# Autodesk Inventor assembly: MeasurementChamber RollBase V1
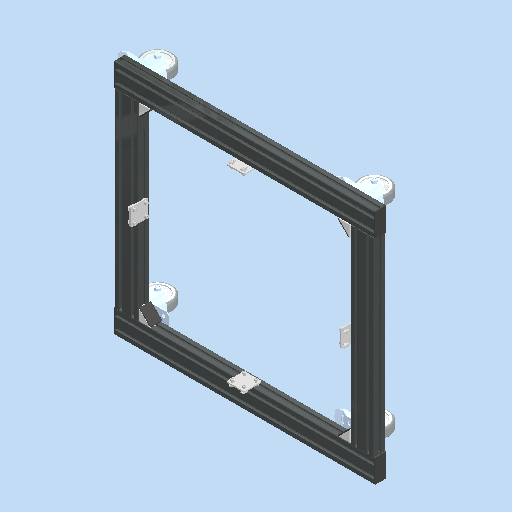
[picture p0: Inventor's stored thumbnail of the model, 512x512]
Saved by Autodesk Inventor 2023.2 (Build 272271000, 271)
## iProperties
Created: 2024-02-20
Part Number: MeasurementChamber RollBase V1
Document SubType Name: Assembly
Designer: Nils Bade
Author: Nils Bade
## Documents named in this file (10)
- C:\Users\nilsb\Documents\Inventor\Projektarbeit-Bade\RatRig_Bade\MeasurementChamber RollBase V1.iam
- C:\Users\nilsb\Documents\Inventor\Projektarbeit-Bade\ITEM\4040 Profile\ITEM T-SLOT 8040 875mm_65530.ipt
- C:\Users\nilsb\Documents\Inventor\Projektarbeit-Bade\ITEM\ITEM_41115_Winkelsatz_90er.iam
- C:\Users\nilsb\Documents\Inventor\Projektarbeit-Bade\ITEM\ITEM Bausätze\ITEM_66718_Lenkrolle-d100-doppelfest.iam
- ITEM_66718_Lenkrolle-d100-doppelfest.iam
- C:\Users\nilsb\Documents\Inventor\Projektarbeit-Bade\ITEM\ITEM Bausätze\ITEM_67018_Befestigungssatz.iam
- ITEM_Befestigungssatz_67018.iam
- C:\Users\nilsb\Documents\Inventor\Projektarbeit-Bade\ITEM\ITEM_Abdeckkappe-80x40-schw_2602.ipt
- C:\Users\nilsb\Documents\Inventor\Projektarbeit-Bade\ITEM\4040 Profile\ITEM T-SLOT 8040 640mm_65530.ipt
- C:\Users\nilsb\Documents\Inventor\Projektarbeit-Bade\RatRig_modified\Base Profile-Connector-Plate - Assembly.iam
## Components (32 placed, 7 different names)
1. ITEM T-SLOT 8040 875mm_65530:1 — Passend:4, Passend:5, Fluchtend:7, Passend:8, Passend:9, Passend:10, Passend:16, Passend:18, Passend:23, Passend:24, Winkel:7, Winkel:8, Winkel:9, Winkel:10, Winkel:11, Winkel:12, Passend:60, Fluchtend:17, Fluchtend:18, Fluchtend:19, Fluchtend:20, Passend:61, Passend:63, Fluchtend:24, Passend:66, Passend:67, Fluchtend:26, Fluchtend:27, Fluchtend:28, Fluchtend:75, Passend:74, Passend:76
2. ITEM T-SLOT 8040 875mm_65530:2 — Passend:6, Passend:7, Passend:11, Passend:14, Passend:19, Passend:22, Passend:25, Winkel:1, Winkel:2, Winkel:3, Winkel:4, Winkel:5, Winkel:6, Fluchtend:15, Fluchtend:16, Passend:59, Fluchtend:21, Fluchtend:22, Passend:62, Fluchtend:23, Passend:64, Fluchtend:25, Fluchtend:29, Passend:71, Fluchtend:78
3. ITEM T-SLOT 8040 640mm_65530:1 — Fluchtend:23, Passend:63, Passend:64, Fluchtend:24, Fluchtend:25, Passend:65, Fluchtend:28, Passend:70, Fluchtend:76, Passend:75, Fluchtend:77
4. ITEM T-SLOT 8040 640mm_65530:2 — Passend:66, Passend:67, Fluchtend:26, Fluchtend:27, Passend:68, Passend:69, Passend:72, Passend:73, Fluchtend:79
5. ITEM_Abdeckkappe-80x40-schw_2602:1 — Fluchtend:21, Fluchtend:22, Passend:62
6. ITEM_Abdeckkappe-80x40-schw_2602:2 — Fluchtend:19, Fluchtend:20, Passend:61
7. ITEM_Abdeckkappe-80x40-schw_2602:3 — Fluchtend:15, Fluchtend:16, Passend:59
8. ITEM_Abdeckkappe-80x40-schw_2602:4 — Passend:60, Fluchtend:17, Fluchtend:18
9. ITEM_41115_Winkelsatz_90er:1 [sub-assembly] — Passend:7, Passend:14, Passend:69
10. ITEM_41115_Winkelsatz_90er:2 [sub-assembly] — Passend:8, Passend:16, Passend:68
11. ITEM_41115_Winkelsatz_90er:3 [sub-assembly] — Passend:9, Passend:10, Passend:70
12. ITEM_41115_Winkelsatz_90er:4 [sub-assembly] — Passend:6, Passend:11, Passend:65
13. Base Profile-Connector-Plate - Assembly:1 [sub-assembly] — Fluchtend:76, Passend:75, Fluchtend:77
14. Base Profile-Connector-Plate - Assembly:2 [sub-assembly] — Fluchtend:75, Passend:74, Passend:76
15. Base Profile-Connector-Plate - Assembly:3 [sub-assembly] — Passend:72, Passend:73, Fluchtend:79
16. Base Profile-Connector-Plate - Assembly:4 [sub-assembly] — Fluchtend:29, Passend:71, Fluchtend:78
17. ITEM_66718_Lenkrolle-d100-doppelfest:1 [sub-assembly] — Passend:18, Fluchtend:8, Fluchtend:10, Passend:24, Passend:41, Passend:42, Passend:43, Passend:44, Passend:45, Passend:46
18. ITEM_66718_Lenkrolle-d100-doppelfest:2 [sub-assembly] — Passend:19, Fluchtend:9, Fluchtend:10, Passend:25, Passend:26, Passend:27, Passend:28, Passend:32, Passend:33, Passend:34
19. ITEM_66718_Lenkrolle-d100-doppelfest:3 [sub-assembly] — Fluchtend:9, Fluchtend:11, Passend:22, Passend:29, Passend:30, Passend:31, Passend:35, Passend:36, Passend:37
20. ITEM_66718_Lenkrolle-d100-doppelfest:4 [sub-assembly] — Fluchtend:8, Fluchtend:11, Passend:23, Passend:38, Passend:39, Passend:40, Passend:47, Passend:48, Passend:49
21. ITEM_Befestigungssatz_67018:1 [sub-assembly] — Passend:41, Winkel:10, Passend:46
22. ITEM_Befestigungssatz_67018:2 [sub-assembly] — Passend:42, Winkel:11, Passend:45
23. ITEM_Befestigungssatz_67018:3 [sub-assembly] — Passend:43, Winkel:12, Passend:44
24. ITEM_Befestigungssatz_67018:4 [sub-assembly] — Passend:38, Winkel:7, Passend:49
25. ITEM_Befestigungssatz_67018:5 [sub-assembly] — Passend:40, Winkel:9, Passend:47
26. ITEM_Befestigungssatz_67018:6 [sub-assembly] — Passend:39, Winkel:8, Passend:48
27. ITEM_Befestigungssatz_67018:7 [sub-assembly] — Passend:30, Winkel:1, Passend:35
28. ITEM_Befestigungssatz_67018:8 [sub-assembly] — Passend:29, Winkel:2, Passend:37
29. ITEM_Befestigungssatz_67018:9 [sub-assembly] — Passend:31, Winkel:3, Passend:36
30. ITEM_Befestigungssatz_67018:10 [sub-assembly] — Passend:28, Winkel:6, Passend:34
31. ITEM_Befestigungssatz_67018:11 [sub-assembly] — Passend:26, Winkel:5, Passend:33
32. ITEM_Befestigungssatz_67018:12 [sub-assembly] — Passend:27, Winkel:4, Passend:32
## Relationships (95: Mate 58, Flush 25, Angle 12)
- Passend:4 [Mate]: ITEM T-SLOT 8040 875mm_65530:1
- Passend:5 [Mate]: ITEM T-SLOT 8040 875mm_65530:1
- Fluchtend:7 [Flush]: ITEM T-SLOT 8040 875mm_65530:1
- Passend:6 [Mate]: ITEM T-SLOT 8040 875mm_65530:2 ↔ ITEM_41115_Winkelsatz_90er:4
- Passend:7 [Mate]: ITEM T-SLOT 8040 875mm_65530:2 ↔ ITEM_41115_Winkelsatz_90er:1
- Passend:8 [Mate]: ITEM T-SLOT 8040 875mm_65530:1 ↔ ITEM_41115_Winkelsatz_90er:2
- Passend:9 [Mate]: ITEM T-SLOT 8040 875mm_65530:1 ↔ ITEM_41115_Winkelsatz_90er:3
- Passend:10 [Mate]: ITEM T-SLOT 8040 875mm_65530:1 ↔ ITEM_41115_Winkelsatz_90er:3
- Passend:11 [Mate]: ITEM T-SLOT 8040 875mm_65530:2 ↔ ITEM_41115_Winkelsatz_90er:4
- Passend:14 [Mate]: ITEM T-SLOT 8040 875mm_65530:2 ↔ ITEM_41115_Winkelsatz_90er:1
- Passend:16 [Mate]: ITEM T-SLOT 8040 875mm_65530:1 ↔ ITEM_41115_Winkelsatz_90er:2
- Passend:18 [Mate] (-20 mm): ITEM T-SLOT 8040 875mm_65530:1 ↔ ITEM_66718_Lenkrolle-d100-doppelfest:1
- Fluchtend:8 [Flush]: ITEM_66718_Lenkrolle-d100-doppelfest:1 ↔ ITEM_66718_Lenkrolle-d100-doppelfest:4
- Passend:19 [Mate] (20 mm): ITEM T-SLOT 8040 875mm_65530:2 ↔ ITEM_66718_Lenkrolle-d100-doppelfest:2
- Fluchtend:9 [Flush]: ITEM_66718_Lenkrolle-d100-doppelfest:2 ↔ ITEM_66718_Lenkrolle-d100-doppelfest:3
- Fluchtend:10 [Flush]: ITEM_66718_Lenkrolle-d100-doppelfest:1 ↔ ITEM_66718_Lenkrolle-d100-doppelfest:2
- Fluchtend:11 [Flush]: ITEM_66718_Lenkrolle-d100-doppelfest:3 ↔ ITEM_66718_Lenkrolle-d100-doppelfest:4
- Passend:22 [Mate]: ITEM T-SLOT 8040 875mm_65530:2 ↔ ITEM_66718_Lenkrolle-d100-doppelfest:3
- Passend:23 [Mate]: ITEM T-SLOT 8040 875mm_65530:1 ↔ ITEM_66718_Lenkrolle-d100-doppelfest:4
- Passend:24 [Mate]: ITEM T-SLOT 8040 875mm_65530:1 ↔ ITEM_66718_Lenkrolle-d100-doppelfest:1
- Passend:25 [Mate]: ITEM T-SLOT 8040 875mm_65530:2 ↔ ITEM_66718_Lenkrolle-d100-doppelfest:2
- Passend:26 [Mate]: ITEM_66718_Lenkrolle-d100-doppelfest:2 ↔ ITEM_Befestigungssatz_67018:11
- Passend:27 [Mate]: ITEM_66718_Lenkrolle-d100-doppelfest:2 ↔ ITEM_Befestigungssatz_67018:12
- Passend:28 [Mate]: ITEM_66718_Lenkrolle-d100-doppelfest:2 ↔ ITEM_Befestigungssatz_67018:10
- Passend:29 [Mate]: ITEM_66718_Lenkrolle-d100-doppelfest:3 ↔ ITEM_Befestigungssatz_67018:8
- Passend:30 [Mate]: ITEM_66718_Lenkrolle-d100-doppelfest:3 ↔ ITEM_Befestigungssatz_67018:7
- Passend:31 [Mate]: ITEM_66718_Lenkrolle-d100-doppelfest:3 ↔ ITEM_Befestigungssatz_67018:9
- Winkel:1 [Angle] (0 deg): ITEM T-SLOT 8040 875mm_65530:2 ↔ ITEM_Befestigungssatz_67018:7
- Winkel:2 [Angle] (0 deg): ITEM T-SLOT 8040 875mm_65530:2 ↔ ITEM_Befestigungssatz_67018:8
- Winkel:3 [Angle] (0 deg): ITEM T-SLOT 8040 875mm_65530:2 ↔ ITEM_Befestigungssatz_67018:9
- Winkel:4 [Angle] (0 deg): ITEM T-SLOT 8040 875mm_65530:2 ↔ ITEM_Befestigungssatz_67018:12
- Winkel:5 [Angle] (0 deg): ITEM T-SLOT 8040 875mm_65530:2 ↔ ITEM_Befestigungssatz_67018:11
- Winkel:6 [Angle] (0 deg): ITEM T-SLOT 8040 875mm_65530:2 ↔ ITEM_Befestigungssatz_67018:10
- Passend:32 [Mate]: ITEM_66718_Lenkrolle-d100-doppelfest:2 ↔ ITEM_Befestigungssatz_67018:12
- Passend:33 [Mate]: ITEM_66718_Lenkrolle-d100-doppelfest:2 ↔ ITEM_Befestigungssatz_67018:11
- Passend:34 [Mate]: ITEM_66718_Lenkrolle-d100-doppelfest:2 ↔ ITEM_Befestigungssatz_67018:10
- Passend:35 [Mate]: ITEM_66718_Lenkrolle-d100-doppelfest:3 ↔ ITEM_Befestigungssatz_67018:7
- Passend:36 [Mate]: ITEM_66718_Lenkrolle-d100-doppelfest:3 ↔ ITEM_Befestigungssatz_67018:9
- Passend:37 [Mate]: ITEM_66718_Lenkrolle-d100-doppelfest:3 ↔ ITEM_Befestigungssatz_67018:8
- Passend:38 [Mate]: ITEM_66718_Lenkrolle-d100-doppelfest:4 ↔ ITEM_Befestigungssatz_67018:4
- Passend:39 [Mate]: ITEM_66718_Lenkrolle-d100-doppelfest:4 ↔ ITEM_Befestigungssatz_67018:6
- Passend:40 [Mate]: ITEM_66718_Lenkrolle-d100-doppelfest:4 ↔ ITEM_Befestigungssatz_67018:5
- Passend:41 [Mate]: ITEM_66718_Lenkrolle-d100-doppelfest:1 ↔ ITEM_Befestigungssatz_67018:1
- Passend:42 [Mate]: ITEM_66718_Lenkrolle-d100-doppelfest:1 ↔ ITEM_Befestigungssatz_67018:2
- Passend:43 [Mate]: ITEM_66718_Lenkrolle-d100-doppelfest:1 ↔ ITEM_Befestigungssatz_67018:3
- Winkel:7 [Angle] (0 deg): ITEM T-SLOT 8040 875mm_65530:1 ↔ ITEM_Befestigungssatz_67018:4
- Winkel:8 [Angle] (0 deg): ITEM T-SLOT 8040 875mm_65530:1 ↔ ITEM_Befestigungssatz_67018:6
- Winkel:9 [Angle] (0 deg): ITEM T-SLOT 8040 875mm_65530:1 ↔ ITEM_Befestigungssatz_67018:5
- Winkel:10 [Angle] (0 deg): ITEM T-SLOT 8040 875mm_65530:1 ↔ ITEM_Befestigungssatz_67018:1
- Winkel:11 [Angle] (0 deg): ITEM T-SLOT 8040 875mm_65530:1 ↔ ITEM_Befestigungssatz_67018:2
- Winkel:12 [Angle] (0 deg): ITEM T-SLOT 8040 875mm_65530:1 ↔ ITEM_Befestigungssatz_67018:3
- Passend:44 [Mate]: ITEM_66718_Lenkrolle-d100-doppelfest:1 ↔ ITEM_Befestigungssatz_67018:3
- Passend:45 [Mate]: ITEM_66718_Lenkrolle-d100-doppelfest:1 ↔ ITEM_Befestigungssatz_67018:2
- Passend:46 [Mate]: ITEM_66718_Lenkrolle-d100-doppelfest:1 ↔ ITEM_Befestigungssatz_67018:1
- Passend:47 [Mate]: ITEM_66718_Lenkrolle-d100-doppelfest:4 ↔ ITEM_Befestigungssatz_67018:5
- Passend:48 [Mate]: ITEM_66718_Lenkrolle-d100-doppelfest:4 ↔ ITEM_Befestigungssatz_67018:6
- Passend:49 [Mate]: ITEM_66718_Lenkrolle-d100-doppelfest:4 ↔ ITEM_Befestigungssatz_67018:4
- Fluchtend:15 [Flush]: ITEM T-SLOT 8040 875mm_65530:2 ↔ ITEM_Abdeckkappe-80x40-schw_2602:3
- Fluchtend:16 [Flush]: ITEM T-SLOT 8040 875mm_65530:2 ↔ ITEM_Abdeckkappe-80x40-schw_2602:3
- Passend:59 [Mate]: ITEM T-SLOT 8040 875mm_65530:2 ↔ ITEM_Abdeckkappe-80x40-schw_2602:3
- Passend:60 [Mate]: ITEM T-SLOT 8040 875mm_65530:1 ↔ ITEM_Abdeckkappe-80x40-schw_2602:4
- Fluchtend:17 [Flush]: ITEM T-SLOT 8040 875mm_65530:1 ↔ ITEM_Abdeckkappe-80x40-schw_2602:4
- Fluchtend:18 [Flush]: ITEM T-SLOT 8040 875mm_65530:1 ↔ ITEM_Abdeckkappe-80x40-schw_2602:4
- Fluchtend:19 [Flush]: ITEM T-SLOT 8040 875mm_65530:1 ↔ ITEM_Abdeckkappe-80x40-schw_2602:2
- Fluchtend:20 [Flush]: ITEM T-SLOT 8040 875mm_65530:1 ↔ ITEM_Abdeckkappe-80x40-schw_2602:2
- Passend:61 [Mate]: ITEM T-SLOT 8040 875mm_65530:1 ↔ ITEM_Abdeckkappe-80x40-schw_2602:2
- Fluchtend:21 [Flush]: ITEM T-SLOT 8040 875mm_65530:2 ↔ ITEM_Abdeckkappe-80x40-schw_2602:1
- Fluchtend:22 [Flush]: ITEM T-SLOT 8040 875mm_65530:2 ↔ ITEM_Abdeckkappe-80x40-schw_2602:1
- Passend:62 [Mate]: ITEM T-SLOT 8040 875mm_65530:2 ↔ ITEM_Abdeckkappe-80x40-schw_2602:1
- Fluchtend:23 [Flush]: ITEM T-SLOT 8040 875mm_65530:2 ↔ ITEM T-SLOT 8040 640mm_65530:1
- Passend:63 [Mate]: ITEM T-SLOT 8040 875mm_65530:1 ↔ ITEM T-SLOT 8040 640mm_65530:1
- Passend:64 [Mate]: ITEM T-SLOT 8040 875mm_65530:2 ↔ ITEM T-SLOT 8040 640mm_65530:1
- Fluchtend:24 [Flush]: ITEM T-SLOT 8040 875mm_65530:1 ↔ ITEM T-SLOT 8040 640mm_65530:1
- Fluchtend:25 [Flush]: ITEM T-SLOT 8040 875mm_65530:2 ↔ ITEM T-SLOT 8040 640mm_65530:1
- Passend:65 [Mate]: ITEM T-SLOT 8040 640mm_65530:1 ↔ ITEM_41115_Winkelsatz_90er:4
- Passend:66 [Mate]: ITEM T-SLOT 8040 875mm_65530:1 ↔ ITEM T-SLOT 8040 640mm_65530:2
- Passend:67 [Mate]: ITEM T-SLOT 8040 875mm_65530:1 ↔ ITEM T-SLOT 8040 640mm_65530:2
- Fluchtend:26 [Flush]: ITEM T-SLOT 8040 875mm_65530:1 ↔ ITEM T-SLOT 8040 640mm_65530:2
- Fluchtend:27 [Flush]: ITEM T-SLOT 8040 875mm_65530:1 ↔ ITEM T-SLOT 8040 640mm_65530:2
- Passend:68 [Mate]: ITEM T-SLOT 8040 640mm_65530:2 ↔ ITEM_41115_Winkelsatz_90er:2
- Passend:69 [Mate]: ITEM T-SLOT 8040 640mm_65530:2 ↔ ITEM_41115_Winkelsatz_90er:1
- Fluchtend:28 [Flush]: ITEM T-SLOT 8040 875mm_65530:1 ↔ ITEM T-SLOT 8040 640mm_65530:1
- Passend:70 [Mate]: ITEM T-SLOT 8040 640mm_65530:1 ↔ ITEM_41115_Winkelsatz_90er:3
- Fluchtend:29 [Flush]: ITEM T-SLOT 8040 875mm_65530:2 ↔ Base Profile-Connector-Plate - Assembly:4
- Passend:71 [Mate]: ITEM T-SLOT 8040 875mm_65530:2 ↔ Base Profile-Connector-Plate - Assembly:4
- Passend:72 [Mate]: ITEM T-SLOT 8040 640mm_65530:2 ↔ Base Profile-Connector-Plate - Assembly:3
- Passend:73 [Mate]: ITEM T-SLOT 8040 640mm_65530:2 ↔ Base Profile-Connector-Plate - Assembly:3
- Fluchtend:75 [Flush]: ITEM T-SLOT 8040 875mm_65530:1 ↔ Base Profile-Connector-Plate - Assembly:2
- Passend:74 [Mate]: ITEM T-SLOT 8040 875mm_65530:1 ↔ Base Profile-Connector-Plate - Assembly:2
- Fluchtend:76 [Flush]: ITEM T-SLOT 8040 640mm_65530:1 ↔ Base Profile-Connector-Plate - Assembly:1
- Passend:75 [Mate]: ITEM T-SLOT 8040 640mm_65530:1 ↔ Base Profile-Connector-Plate - Assembly:1
- Fluchtend:77 [Flush]: ITEM T-SLOT 8040 640mm_65530:1 ↔ Base Profile-Connector-Plate - Assembly:1
- Passend:76 [Mate]: ITEM T-SLOT 8040 875mm_65530:1 ↔ Base Profile-Connector-Plate - Assembly:2
- Fluchtend:78 [Flush]: ITEM T-SLOT 8040 875mm_65530:2 ↔ Base Profile-Connector-Plate - Assembly:4
- Fluchtend:79 [Flush]: ITEM T-SLOT 8040 640mm_65530:2 ↔ Base Profile-Connector-Plate - Assembly:3
